# Autodesk Inventor assembly: Муфта 30мм
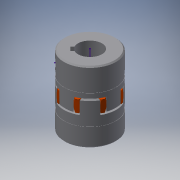
[picture p0: Inventor's stored thumbnail of the model, 180x180]
Saved by Autodesk Inventor 2016 (Build 200138000, 138)
## iProperties
Created: 2021-04-30
Part Number: Муфта 30мм
Material: Типовые
Document SubType Name: Assembly
Designer: Лол
Author: Лол
## Documents named in this file (4)
- C:\Users\Лол\Documents\Inventor\course_work\Муфта 30мм.iam
- C:\Users\Лол\Documents\Inventor\course_work\Муфта резинка 30мм.ipt
- C:\Users\Лол\Documents\Inventor\course_work\Муфта железка 30мм.ipt
- C:\Users\Лол\Documents\Inventor\course_work\AS 1421 - M8x12 конический.ipt
## Components (5 placed, 3 different names)
1. Муфта железка 30мм:1 — Совмещение:1, Совмещение:2, Совмещение:4, Угол:1, Совмещение:6
2. Муфта железка 30мм:2 — Совмещение:3, Совмещение:4, Угол:1, Угол:2, Совмещение:5
3. Муфта резинка 30мм:1 — Совмещение:1, Совмещение:2, Совмещение:3, Угол:2
4. AS 1421 - M8x12 конический:1 — Совмещение:5
5. AS 1421 - M8x12 конический:2 — Совмещение:6
## Relationships (8: Mate 6, Angle 2)
- Совмещение:1 [Mate]: Муфта железка 30мм:1 ↔ Муфта резинка 30мм:1
- Совмещение:2 [Mate]: Муфта железка 30мм:1 ↔ Муфта резинка 30мм:1
- Совмещение:3 [Mate]: Муфта железка 30мм:2 ↔ Муфта резинка 30мм:1
- Совмещение:4 [Mate]: Муфта железка 30мм:1 ↔ Муфта железка 30мм:2
- Угол:1 [Angle] (45 deg): Муфта железка 30мм:1 ↔ Муфта железка 30мм:2
- Угол:2 [Angle] (22.5 deg): Муфта железка 30мм:2 ↔ Муфта резинка 30мм:1
- Совмещение:5 [Mate]: Муфта железка 30мм:2 ↔ AS 1421 - M8x12 конический:1
- Совмещение:6 [Mate]: Муфта железка 30мм:1 ↔ AS 1421 - M8x12 конический:2
